# Autodesk Inventor assembly: PrzyciskSTOP
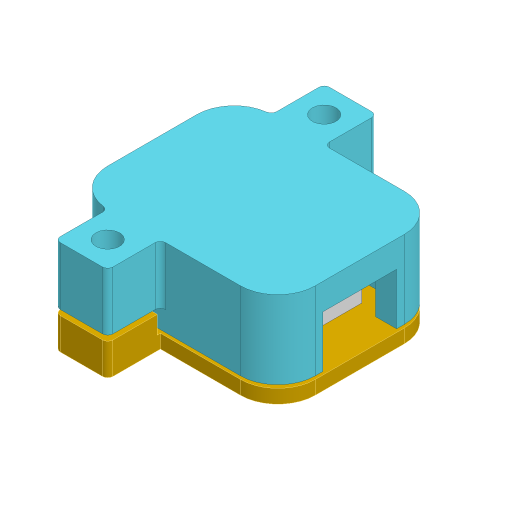
[picture p0: Inventor's stored thumbnail of the model, 512x512]
Saved by Autodesk Inventor 2024.3 (Build 283343000, 343)
## iProperties
Created: 2025-08-19
Part Number: PrzyciskSTOP
Document SubType Name: Assembly
Designer: PM
Author: PM
## Documents named in this file (4)
- C:\MPA - shortPath\magisterka\V3\Workspace\PrzyciskSTOP.iam
- C:\MPA - shortPath\magisterka\V3\Workspace\DF Robot DFR0029-R.ipt
- C:\MPA - shortPath\magisterka\V3\Workspace\PrzyciskSTOP_1.ipt
- C:\MPA - shortPath\magisterka\V3\Workspace\PrzyciskSTOP_2.ipt
## Components (3 placed, 3 different names)
1. DF Robot DFR0029-R:1 — Flush:1, Flush:2, Flush:3, Flush:4
2. PrzyciskSTOP_1:1 — Flush:4, Flush:5
3. PrzyciskSTOP_2:1 — Flush:5
## Relationships (5: Flush 5)
- Flush:1: DF Robot DFR0029-R:1
- Flush:2: DF Robot DFR0029-R:1
- Flush:3: DF Robot DFR0029-R:1
- Flush:4: DF Robot DFR0029-R:1 ↔ PrzyciskSTOP_1:1
- Flush:5: PrzyciskSTOP_1:1 ↔ PrzyciskSTOP_2:1
